# Autodesk Inventor assembly: Robot
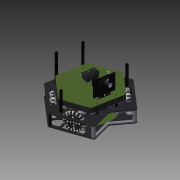
[picture p0: Inventor's stored thumbnail of the model, 180x180]
Saved by Autodesk Inventor 2015 (Build 190159000, 159)
## iProperties
Created: 2016-10-01
Part Number: Robot
Document SubType Name: Assembly
Designer: James Yelland
Author: James Yelland
## Documents named in this file (21)
- C:\Users\James Yelland\git\LJ-STAND\Design\Models\Version 2\Robot.iam
- C:\Users\James Yelland\git\LJ-STAND\Design\Models\Version 2\Bottom Plate.ipt
- C:\Users\James Yelland\git\LJ-STAND\Design\Models\Version 2\Middle Plate.ipt
- C:\Users\James Yelland\git\LJ-STAND\Design\Models\Common\Standoff 30.ipt
- C:\Users\James Yelland\git\LJ-STAND\Design\Models\Version 2\Motor Mount.ipt
- C:\Users\James Yelland\git\LJ-STAND\Design\Models\Common\Standoff 10.ipt
- C:\Users\James Yelland\git\LJ-STAND\Design\Models\Version 2\PCB.ipt
- C:\Users\James Yelland\git\LJ-STAND\Design\Models\Version 2\TSOP Cover Ring.ipt
- C:\Users\James Yelland\git\LJ-STAND\Design\Models\Version 2\Light Sensor PCB.ipt
- C:\Users\James Yelland\git\LJ-STAND\Design\Models\Version 2\Top Plate.ipt
- C:\Users\James Yelland\git\LJ-STAND\Design\Models\Common\Standoff 20.ipt
- C:\Users\James Yelland\git\LJ-STAND\Design\Models\Version 2\Handle.ipt
- C:\Users\James Yelland\git\LJ-STAND\Design\Models\Common\Standoff 50.ipt
- C:\Users\James Yelland\git\LJ-STAND\Design\Models\Pixy\pixy\Imported Components\Pixy(CMUcam5)\Pixy(CMUcam5).iam
- C:\Users\James Yelland\git\LJ-STAND\Design\Models\Wheel\Wheel.iam
- C:\Users\James Yelland\git\LJ-STAND\Design\Models\Common\Toggle switch.ipt
- C:\Users\James Yelland\git\LJ-STAND\Design\Models\Common\Battery.ipt
- C:\Users\James Yelland\git\LJ-STAND\Design\Models\Common\Pixy angle bracket.ipt
- C:\Users\James Yelland\git\LJ-STAND\Design\Models\Common\Imported Components\maxon_PN_0_1\maxon_PN_0_1.iam
- C:\Users\James Yelland\git\LJ-STAND\Design\Models\Version 2\Motor Support.ipt
- C:\Users\James Yelland\git\LJ-STAND\Design\Models\Version 2\Front mount.ipt
## Components (41 placed, 20 different names)
1. Bottom Plate:1 — Mate:1, Mate:2, Mate:3, Mate:4, Mate:5, Mate:6, Mate:7, Mate:8, Mate:12, Mate:13, Mate:14, Mate:15, Mate:16, Mate:17, Mate:70, Mate:71, Mate:72, Mate:76, Mate:77, Mate:78, Insert:40, Insert:41, Insert:46, Insert:47, Insert:48
2. Middle Plate:1 — Mate:9, Mate:10, Mate:11, Mate:61, Mate:62, Insert:1, Insert:2, Insert:3, Insert:4, Insert:18, Insert:19, Insert:20, Insert:21, Insert:26, Insert:27, Mate:93, Flush:5, Insert:49
3. Standoff 30:1 — Mate:4, Mate:5
4. Standoff 30:2 — Mate:3, Mate:6, Mate:9, Mate:11
5. Standoff 30:3 — Mate:2, Mate:8
6. Standoff 30:4 — Mate:1, Mate:7, Mate:10, Mate:94
7. Motor Mount:1 — Mate:12, Mate:13, Mate:14, Mate:86, Insert:44
8. Motor Mount:2 — Mate:15, Mate:16, Mate:17, Mate:84, Insert:42
9. Standoff 10:1 — Mate:61, Insert:4
10. Standoff 10:2 — Insert:2, Insert:15
11. Standoff 10:3 — Insert:1, Insert:14
12. Standoff 10:4 — Mate:62, Insert:3
13. Light Sensor PCB:1 — Insert:40, Insert:41
14. Top Plate:1 — Insert:10, Insert:11, Insert:22, Insert:23, Mate:87, Mate:88, Mate:89, Mate:90, Mate:91, Mate:92
15. Standoff 20:1 — Insert:10, Insert:12
16. Standoff 20:2 — Insert:11, Insert:13
17. Handle:1 — Insert:12, Insert:13
18. TSOP Cover Ring:1 — Insert:14, Insert:15, Insert:16, Insert:17, Angle:1, Angle:2
19. PCB:1 — Insert:16, Insert:17, Insert:36, Insert:37
20. Standoff 50:1 — Insert:19, Insert:23
21. Standoff 50:2 — Insert:18, Insert:22
22. Standoff 50:3 — Insert:21, Insert:27
23. Standoff 50:4 — Insert:20, Insert:26
24. Pixy(CMUcam5):1 [sub-assembly] — Insert:38, Insert:39
25. Motor Mount:3 — Mate:76, Mate:77, Mate:78, Mate:85, Insert:43
26. Motor Mount:4 — Mate:70, Mate:71, Mate:72, Mate:80, Insert:45
27. Wheel:1 [sub-assembly] — Mate:84, Mate:96
28. Wheel:2 [sub-assembly] — Mate:85, Mate:97
29. Wheel:3 [sub-assembly] — Mate:86, Mate:95
30. Wheel:4 [sub-assembly] — Mate:80, Mate:98
31. Toggle switch:1 — Mate:90, Mate:91, Mate:92
32. Toggle switch:2 — Mate:87, Mate:88, Mate:89
33. Battery:1 — Mate:93, Flush:5, Mate:94
34. Pixy angle bracket:1 — Insert:36, Angle:2, Insert:38
35. Pixy angle bracket:2 — Insert:37, Angle:1, Insert:39
36. maxon_PN_0_1:1 [sub-assembly] — Insert:42, Mate:96
37. maxon_PN_0_1:2 [sub-assembly] — Insert:44, Mate:95
38. maxon_PN_0_1:3 [sub-assembly] — Insert:45, Mate:98
39. maxon_PN_0_1:4 [sub-assembly] — Insert:43, Mate:97
40. Motor Support:1 — Insert:46, Insert:47
41. Front mount:1 — Insert:48, Insert:49
## Relationships (78: Mate 41, Insert 34, Angle 2, Flush 1)
- Mate:1: Bottom Plate:1 ↔ Standoff 30:4
- Mate:2: Bottom Plate:1 ↔ Standoff 30:3
- Mate:3: Bottom Plate:1 ↔ Standoff 30:2
- Mate:4: Bottom Plate:1 ↔ Standoff 30:1
- Mate:5: Bottom Plate:1 ↔ Standoff 30:1
- Mate:6: Bottom Plate:1 ↔ Standoff 30:2
- Mate:7: Bottom Plate:1 ↔ Standoff 30:4
- Mate:8: Bottom Plate:1 ↔ Standoff 30:3
- Mate:9: Middle Plate:1 ↔ Standoff 30:2
- Mate:10: Middle Plate:1 ↔ Standoff 30:4
- Mate:11: Middle Plate:1 ↔ Standoff 30:2
- Mate:12: Bottom Plate:1 ↔ Motor Mount:1
- Mate:13: Bottom Plate:1 ↔ Motor Mount:1
- Mate:14: Bottom Plate:1 ↔ Motor Mount:1
- Mate:15: Bottom Plate:1 ↔ Motor Mount:2
- Mate:16: Bottom Plate:1 ↔ Motor Mount:2
- Mate:17: Bottom Plate:1 ↔ Motor Mount:2
- Mate:61: Middle Plate:1 ↔ Standoff 10:1
- Mate:62: Middle Plate:1 ↔ Standoff 10:4
- Insert:1: Middle Plate:1 ↔ Standoff 10:3
- Insert:2: Middle Plate:1 ↔ Standoff 10:2
- Insert:3: Middle Plate:1 ↔ Standoff 10:4
- Insert:4: Middle Plate:1 ↔ Standoff 10:1
- Insert:10: Top Plate:1 ↔ Standoff 20:1
- Insert:11: Top Plate:1 ↔ Standoff 20:2
- Insert:12: Standoff 20:1 ↔ Handle:1
- Insert:13: Standoff 20:2 ↔ Handle:1
- Insert:14: Standoff 10:3 ↔ TSOP Cover Ring:1
- Insert:15: Standoff 10:2 ↔ TSOP Cover Ring:1
- Insert:16: TSOP Cover Ring:1 ↔ PCB:1
- Insert:17: TSOP Cover Ring:1 ↔ PCB:1
- Insert:18: Middle Plate:1 ↔ Standoff 50:2
- Insert:19: Middle Plate:1 ↔ Standoff 50:1
- Insert:20: Middle Plate:1 ↔ Standoff 50:4
- Insert:21: Middle Plate:1 ↔ Standoff 50:3
- Insert:22: Top Plate:1 ↔ Standoff 50:2
- Insert:23: Top Plate:1 ↔ Standoff 50:1
- Mate:70: Bottom Plate:1 ↔ Motor Mount:4
- Mate:71: Bottom Plate:1 ↔ Motor Mount:4
- Mate:72: Bottom Plate:1 ↔ Motor Mount:4
- Insert:26: Middle Plate:1 ↔ Standoff 50:4
- Insert:27: Middle Plate:1 ↔ Standoff 50:3
- Mate:76: Bottom Plate:1 ↔ Motor Mount:3
- Mate:77: Bottom Plate:1 ↔ Motor Mount:3
- Mate:78: Bottom Plate:1 ↔ Motor Mount:3
- Mate:80 (5 mm): Motor Mount:4 ↔ Wheel:4
- Mate:84 (5 mm): Motor Mount:2 ↔ Wheel:1
- Mate:85 (5 mm): Motor Mount:3 ↔ Wheel:2
- Mate:86 (5 mm): Motor Mount:1 ↔ Wheel:3
- Mate:87: Top Plate:1 ↔ Toggle switch:2
- Mate:88: Top Plate:1 ↔ Toggle switch:2
- Mate:89: Top Plate:1 ↔ Toggle switch:2
- Mate:90: Top Plate:1 ↔ Toggle switch:1
- Mate:91: Top Plate:1 ↔ Toggle switch:1
- Mate:92: Top Plate:1 ↔ Toggle switch:1
- Mate:93: Middle Plate:1 ↔ Battery:1
- Flush:5 (5 mm): Middle Plate:1 ↔ Battery:1
- Mate:94 (10 mm): Standoff 30:4 ↔ Battery:1
- Insert:36: PCB:1 ↔ Pixy angle bracket:1
- Insert:37: PCB:1 ↔ Pixy angle bracket:2
- Angle:1 (0 deg): TSOP Cover Ring:1 ↔ Pixy angle bracket:2
- Angle:2 (0 deg): TSOP Cover Ring:1 ↔ Pixy angle bracket:1
- Insert:38: Pixy(CMUcam5):1 ↔ Pixy angle bracket:1
- Insert:39: Pixy(CMUcam5):1 ↔ Pixy angle bracket:2
- Insert:40: Bottom Plate:1 ↔ Light Sensor PCB:1
- Insert:41: Bottom Plate:1 ↔ Light Sensor PCB:1
- Insert:42: Motor Mount:2 ↔ maxon_PN_0_1:1
- Insert:43: Motor Mount:3 ↔ maxon_PN_0_1:4
- Insert:44: Motor Mount:1 ↔ maxon_PN_0_1:2
- Insert:45: Motor Mount:4 ↔ maxon_PN_0_1:3
- Mate:95: Wheel:3 ↔ maxon_PN_0_1:2
- Mate:96: Wheel:1 ↔ maxon_PN_0_1:1
- Mate:97: Wheel:2 ↔ maxon_PN_0_1:4
- Mate:98: Wheel:4 ↔ maxon_PN_0_1:3
- Insert:46: Bottom Plate:1 ↔ Motor Support:1
- Insert:47: Bottom Plate:1 ↔ Motor Support:1
- Insert:48: Bottom Plate:1 ↔ Front mount:1
- Insert:49: Middle Plate:1 ↔ Front mount:1
